# Autodesk Inventor assembly: AXIS_DEV_EDT_V3
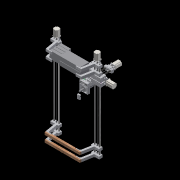
[picture p0: Inventor's stored thumbnail of the model, 180x180]
Saved by Autodesk Inventor 2016 (Build 200138000, 138)
## iProperties
Created: 2017-07-14
Part Number: AXIS_DEV_EDT_V3
Document SubType Name: Assembly
Designer: ludwi
Author: ludwi
## Documents named in this file (19)
- H:\MARQ\3D\AXIS_DEV_EDT_V3\AXIS_DEV_EDT_V3.iam
- H:\MARQ\3D\AXIS_DEV_EDT_V3\Z.iam
- H:\MARQ\3D\AXIS_DEV_EDT_V3\AXCAR.ipt
- H:\MARQ\3D\AXIS_DEV_EDT_V3\Y.iam
- H:\MARQ\3D\AXIS_DEV_EDT_V3\X.iam
- H:\MARQ\3D\AXIS_DEV_EDT_V3\AXTS.ipt
- H:\MARQ\3D\AXIS_DEV_EDT_V3\AXMM.ipt
- H:\MARQ\3D\AXIS_DEV_EDT_V3\AXLG.ipt
- H:\MARQ\3D\AXIS_DEV_EDT_V3\STP_SP.ipt
- H:\MARQ\3D\AXIS_DEV_EDT_V3\STP_DR.ipt
- H:\MARQ\3D\AXIS_DEV_EDT_V3\DNW_CON.ipt
- H:\MARQ\3D\AXIS_DEV_EDT_V3\AXB_HALF.ipt
- H:\MARQ\3D\AXIS_DEV_EDT_V3\AXCAR_HALF.ipt
- H:\MARQ\3D\AXIS_DEV_EDT_V3\SPINDLE.ipt
- H:\MARQ\3D\AXIS_DEV_EDT_V3\DNW_CON_V2.ipt
- H:\MARQ\3D\AXIS_DEV_EDT_V3\AXIS_DEV_EDT_V3\AIP\FEA\c7l11emw0.fins
- H:\MARQ\3D\AXIS_DEV_EDT_V3\AXIS_DEV_EDT_V3\AIP\FEA\c7l11emw0.fsat
- H:\MARQ\3D\AXIS_DEV_EDT_V3\AXIS_DEV_EDT_V3\AIP\FEA\c7l11emw0.ftes
- H:\MARQ\3D\AXIS_DEV_EDT_V3\AXIS_DEV_EDT_V3\AIP\FEA\c7l11emw0.fwiz
## Components (41 placed, 14 different names)
1. X:2 [sub-assembly] — Mate:5, Mate:6, Flush:6, Mate:17, Flush:28, Flush:29, Mate:31, Flush:31, Flush:32, Flush:36, Flush:37, Mate:38, Flush:38
2. AXCAR:3 — Mate:5, Mate:6, Insert:3, Insert:4, Flush:13
3. AXCAR:4 — Insert:3, Insert:4, Flush:25, Insert:15
4. AXLG:1 — Flush:6, Flush:26, Flush:43
5. AXLG:4 — Mate:17, Flush:28, Flush:29
6. X:3 [sub-assembly] — Mate:10, Flush:7, Flush:8, Flush:10, Flush:11, Mate:11, Mate:12, Mate:13, Flush:38, Mate:44, Flush:46
7. AXLG:5 — Mate:10, Flush:7, Flush:8
8. AXLG:6 — Flush:10, Flush:11, Mate:11
9. AXCAR:5 — Mate:12, Mate:13
10. AXCAR:6 — Flush:13, Mate:26, Insert:14
11. Y:1 [sub-assembly] — Mate:14, Mate:15, Flush:25, Mate:26, Insert:14, Insert:15
12. AXCAR:7 — Mate:14, Mate:15, Mate:19, Flush:14, Flush:17
13. AXCAR:8 — Mate:18, Flush:15, Flush:16
14. AXTS:1 — Mate:18, Flush:15, Flush:16, Mate:20, Flush:18, Flush:19, Insert:24, Insert:25
15. AXTS:2 — Mate:19, Flush:14, Flush:17
16. AXCAR:9 — Flush:19
17. AXCAR:10 — Mate:20, Flush:18, Mate:21, Mate:22
18. Z:1 [sub-assembly] — Mate:21, Mate:22, Mate:23, Flush:20, Flush:21, Mate:40, Flush:39, Flush:40
19. AXMM:1 — Mate:23, Flush:20, Flush:21, Flush:22, Flush:23, Mate:24, Mate:39
20. AXMM:2 — Flush:22, Flush:23, Mate:24
21. STP_SP:1
22. STP_SP:2
23. STP_DR:1
24. STP_DR:2
25. STP_DR:3
26. STP_DR:4
27. DNW_CON:1 — Flush:26
28. AXLG:7 — Mate:31, Flush:31, Flush:32
29. AXLG:8
30. AXLG:9 — Flush:36, Flush:37, Mate:38
31. AXLG:10 — Mate:43, Flush:44, Flush:45, Mate:44, Flush:46
32. DNW_CON:4
33. AXB_HALF:1
34. AXCAR_HALF:1 — Insert:24, Insert:25, Insert:26, Insert:27
35. AXCAR_HALF:2 — Insert:26, Insert:27
36. SPINDLE:1 — Mate:39
37. AXMM:3 — Mate:40, Flush:39, Flush:40, Mate:41, Flush:41, Flush:42, Mate:42
38. AXMM:4 — Mate:41, Flush:41, Flush:42
39. SPINDLE:2 — Mate:42
40. DNW_CON_V2:1 — Flush:43
41. DNW_CON_V2:2 — Mate:43, Flush:44, Flush:45
## Relationships (74: Flush 35, Mate 25, Insert 14)
- Mate:5: X:2 ↔ AXCAR:3
- Mate:6: X:2 ↔ AXCAR:3
- Insert:3: AXCAR:3 ↔ AXCAR:4
- Insert:4: AXCAR:3 ↔ AXCAR:4
- Flush:6: X:2 ↔ AXLG:1
- Mate:10: X:3 ↔ AXLG:5
- Flush:7: X:3 ↔ AXLG:5
- Flush:8: X:3 ↔ AXLG:5
- Flush:10: X:3 ↔ AXLG:6
- Flush:11: X:3 ↔ AXLG:6
- Mate:11: X:3 ↔ AXLG:6
- [Insert]: AXCAR:5 ↔ AXCAR:6
- [Insert]: AXCAR:5 ↔ AXCAR:6
- Mate:12: X:3 ↔ AXCAR:5
- Mate:13: X:3 ↔ AXCAR:5
- Flush:13: AXCAR:3 ↔ AXCAR:6
- [Insert]: AXCAR:7 ↔ AXCAR:8
- [Insert]: AXCAR:7 ↔ AXCAR:8
- Mate:14: Y:1 ↔ AXCAR:7
- Mate:15: Y:1 ↔ AXCAR:7
- Mate:17: X:2 ↔ AXLG:4
- Mate:18: AXCAR:8 ↔ AXTS:1
- Mate:19: AXCAR:7 ↔ AXTS:2
- Flush:14: AXCAR:7 ↔ AXTS:2
- Flush:15: AXCAR:8 ↔ AXTS:1
- Flush:16: AXCAR:8 ↔ AXTS:1
- Flush:17: AXCAR:7 ↔ AXTS:2
- [Insert]: AXCAR:9 ↔ AXCAR:10
- [Insert]: AXCAR:9 ↔ AXCAR:10
- Mate:20: AXTS:1 ↔ AXCAR:10
- Flush:18: AXTS:1 ↔ AXCAR:10
- Flush:19: AXTS:1 ↔ AXCAR:9
- Mate:21: AXCAR:10 ↔ Z:1
- Mate:22: AXCAR:10 ↔ Z:1
- Mate:23: Z:1 ↔ AXMM:1
- Flush:20: Z:1 ↔ AXMM:1
- Flush:21: Z:1 ↔ AXMM:1
- Flush:22: AXMM:1 ↔ AXMM:2
- Flush:23: AXMM:1 ↔ AXMM:2
- Mate:24: AXMM:1 ↔ AXMM:2
- Flush:25: AXCAR:4 ↔ Y:1
- Mate:26: AXCAR:6 ↔ Y:1
- Insert:14: AXCAR:6 ↔ Y:1
- Insert:15: AXCAR:4 ↔ Y:1
- Flush:26: AXLG:1 ↔ DNW_CON:1
- Flush:28: X:2 ↔ AXLG:4
- Flush:29: X:2 ↔ AXLG:4
- Mate:31: X:2 ↔ AXLG:7
- Flush:31: X:2 ↔ AXLG:7
- Flush:32: X:2 ↔ AXLG:7
- [Flush]: AXLG:9 ↔ DNW_CON:4
- [Flush]: AXLG:10 ↔ DNW_CON:4
- Flush:36: X:2 ↔ AXLG:9
- Flush:37: X:2 ↔ AXLG:9
- Mate:38: X:2 ↔ AXLG:9
- Flush:38: X:2 ↔ X:3
- Insert:24: AXTS:1 ↔ AXCAR_HALF:1
- Insert:25: AXTS:1 ↔ AXCAR_HALF:1
- Insert:26: AXCAR_HALF:1 ↔ AXCAR_HALF:2
- Insert:27: AXCAR_HALF:1 ↔ AXCAR_HALF:2
- Mate:39: AXMM:1 ↔ SPINDLE:1
- Mate:40: Z:1 ↔ AXMM:3
- Flush:39: Z:1 ↔ AXMM:3
- Flush:40: Z:1 ↔ AXMM:3
- Mate:41: AXMM:3 ↔ AXMM:4
- Flush:41: AXMM:3 ↔ AXMM:4
- Flush:42: AXMM:3 ↔ AXMM:4
- Mate:42: AXMM:3 ↔ SPINDLE:2
- Flush:43: AXLG:1 ↔ DNW_CON_V2:1
- Mate:43: AXLG:10 ↔ DNW_CON_V2:2
- Flush:44: AXLG:10 ↔ DNW_CON_V2:2
- Flush:45: AXLG:10 ↔ DNW_CON_V2:2
- Mate:44: X:3 ↔ AXLG:10
- Flush:46: X:3 ↔ AXLG:10
## Named parameters: sa_0 = -2.8332e-09, sa_1 = 5.39e-11, sa_2 = -10000, d195_d62 = 0 mm, d196_d63 = 0 mm, d203_d62 = 0 mm, d204_d63 = 0 mm, d215_d203_d62 = 0 mm, d216_d204_d63 = 0 mm, d279_d270_d265 = 0 mm, d282_d276 = 0 mm
note: some values were not read from the file. Shown as the stored number, unit unknown: "sa_0", "sa_1", "sa_2".
